# Autodesk Inventor assembly: szafa xD
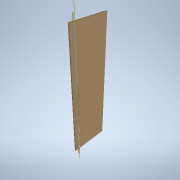
[picture p0: Inventor's stored thumbnail of the model, 180x180]
Saved by Autodesk Inventor 2021 (Build 250183000, 183)
## iProperties
Created: 2021-04-01
Part Number: szafa xD
Document SubType Name: Assembly
Designer: Wojciech Wołczek
Author: Wojciech Wołczek
## Documents named in this file (22)
- D:\OneDrive\Documents\inventor\szafa xD.iam
- D:\OneDrive\Documents\inventor\ISO 10799-2 - 25x25x2.5 - 2000.ipt
- D:\OneDrive\Documents\inventor\sciana.ipt
- D:\Documents\Inventor\Content Center Files\R2021\pl-PL\ANSI_ASME B18.6.5M(7)\ANSI_ASME B18.6.5M - M2,5x0,45 x 4(2) F.ipt
- D:\OneDrive\Documents\inventor\szafa xD\AIP\FEA\dka5v7oqo.fins
- D:\OneDrive\Documents\inventor\szafa xD\AIP\FEA\dka5v7oqo.fsat
- D:\OneDrive\Documents\inventor\szafa xD\AIP\FEA\dka5v7oqo.ftes
- D:\OneDrive\Documents\inventor\szafa xD\AIP\FEA\dka5v7oqo.fwiz
- D:\OneDrive\Documents\inventor\szafa xD\AIP\FEA\dka5v7oqp.fins
- D:\OneDrive\Documents\inventor\szafa xD\AIP\FEA\dka5v7oqp.fsat
- D:\OneDrive\Documents\inventor\szafa xD\AIP\FEA\dka5v7oqp.ftes
- D:\OneDrive\Documents\inventor\szafa xD\AIP\FEA\dka5v7oqp.fwiz
- D:\OneDrive\Documents\inventor\szafa xD\AIP\FEA\dka5v7oqq.fins
- D:\OneDrive\Documents\inventor\szafa xD\AIP\FEA\dka5v7oqq.fsat
- D:\OneDrive\Documents\inventor\szafa xD\AIP\FEA\dka5v7oqq.ftes
- D:\OneDrive\Documents\inventor\szafa xD\AIP\FEA\dka5v7ork.fwiz
- D:\OneDrive\Documents\inventor\szafa xD\AIP\FEA\dka5v7osg.fmsh
- D:\OneDrive\Documents\inventor\szafa xD\AIP\FEA\dka5v7osh.fres
- D:\OneDrive\Documents\inventor\szafa xD\AIP\FEA\dka5v7otc.fmsh
- D:\OneDrive\Documents\inventor\szafa xD\AIP\FEA\dka5v7otd.fres
- D:\OneDrive\Documents\inventor\szafa xD\AIP\FEA\dka5v7ou8.fmsh
- D:\OneDrive\Documents\inventor\szafa xD\AIP\FEA\dka5v7ou9.fres
## Components (78 placed, 3 different names)
1. ISO 10799-2 - 25x25x2.5 - 2000:1 — Równoległe:1, Równoległe:2, Wstawiające:1, Wstawiające:2, Wstawiające:3, Wstawiające:4, Wstawiające:5, Wstawiające:6, Wstawiające:7, Wstawiające:8, Wstawiające:9, Wstawiające:10, Wstawiające:11, Wstawiające:12, Wstawiające:13, Wstawiające:14, Wstawiające:15, Wstawiające:16, Wstawiające:17, Wstawiające:18, Wstawiające:19, Wstawiające:20, Wstawiające:21, Wstawiające:22, Wstawiające:23, Wstawiające:24, Wstawiające:25, Wstawiające:26, Wstawiające:27, Wstawiające:28, Wstawiające:29, Wstawiające:30, Wstawiające:31, Wstawiające:32, Wstawiające:33, Wstawiające:34, Wstawiające:35, Wstawiające:36, Wstawiające:37, Wstawiające:38, Wstawiające:39, Wstawiające:40, Wstawiające:41, Wstawiające:42, Wstawiające:43, Wstawiające:44, Wstawiające:45, Wstawiające:46, Wstawiające:47, Wstawiające:48, Wstawiające:49, Wstawiające:50, Wstawiające:51, Wstawiające:52, Wstawiające:53, Wstawiające:54, Wstawiające:55, Wstawiające:56, Wstawiające:57, Wstawiające:58, Wstawiające:59, Wstawiające:60, Wstawiające:61, Wstawiające:62, Wstawiające:63, Wstawiające:64, Wstawiające:65, Wstawiające:66, Wstawiające:67, Wstawiające:68, Wstawiające:69, Wstawiające:70, Wstawiające:71, Wstawiające:72, Wstawiające:73, Wstawiające:74, Wstawiające:75, Wstawiające:76
2. sciana:1 — Równoległe:1, Równoległe:2
3. Wkręt samogwintujący z łbem walcowym wypukłym z rowkiem prostym - Typ F - Metryczny M2,5x0,45 x 4:1 — Wstawiające:1
4. Wkręt samogwintujący z łbem walcowym wypukłym z rowkiem prostym - Typ F - Metryczny M2,5x0,45 x 4:2 — Wstawiające:2
5. Wkręt samogwintujący z łbem walcowym wypukłym z rowkiem prostym - Typ F - Metryczny M2,5x0,45 x 4:3 — Wstawiające:3
6. Wkręt samogwintujący z łbem walcowym wypukłym z rowkiem prostym - Typ F - Metryczny M2,5x0,45 x 4:4 — Wstawiające:4
7. Wkręt samogwintujący z łbem walcowym wypukłym z rowkiem prostym - Typ F - Metryczny M2,5x0,45 x 4:5 — Wstawiające:5
8. Wkręt samogwintujący z łbem walcowym wypukłym z rowkiem prostym - Typ F - Metryczny M2,5x0,45 x 4:6 — Wstawiające:6
9. Wkręt samogwintujący z łbem walcowym wypukłym z rowkiem prostym - Typ F - Metryczny M2,5x0,45 x 4:7 — Wstawiające:7
10. Wkręt samogwintujący z łbem walcowym wypukłym z rowkiem prostym - Typ F - Metryczny M2,5x0,45 x 4:8 — Wstawiające:8
11. Wkręt samogwintujący z łbem walcowym wypukłym z rowkiem prostym - Typ F - Metryczny M2,5x0,45 x 4:9 — Wstawiające:9
12. Wkręt samogwintujący z łbem walcowym wypukłym z rowkiem prostym - Typ F - Metryczny M2,5x0,45 x 4:10 — Wstawiające:10
13. Wkręt samogwintujący z łbem walcowym wypukłym z rowkiem prostym - Typ F - Metryczny M2,5x0,45 x 4:11 — Wstawiające:11
14. Wkręt samogwintujący z łbem walcowym wypukłym z rowkiem prostym - Typ F - Metryczny M2,5x0,45 x 4:12 — Wstawiające:12
15. Wkręt samogwintujący z łbem walcowym wypukłym z rowkiem prostym - Typ F - Metryczny M2,5x0,45 x 4:13 — Wstawiające:13
16. Wkręt samogwintujący z łbem walcowym wypukłym z rowkiem prostym - Typ F - Metryczny M2,5x0,45 x 4:14 — Wstawiające:14
17. Wkręt samogwintujący z łbem walcowym wypukłym z rowkiem prostym - Typ F - Metryczny M2,5x0,45 x 4:15 — Wstawiające:15
18. Wkręt samogwintujący z łbem walcowym wypukłym z rowkiem prostym - Typ F - Metryczny M2,5x0,45 x 4:16 — Wstawiające:16
19. Wkręt samogwintujący z łbem walcowym wypukłym z rowkiem prostym - Typ F - Metryczny M2,5x0,45 x 4:17 — Wstawiające:17
20. Wkręt samogwintujący z łbem walcowym wypukłym z rowkiem prostym - Typ F - Metryczny M2,5x0,45 x 4:18 — Wstawiające:18
21. Wkręt samogwintujący z łbem walcowym wypukłym z rowkiem prostym - Typ F - Metryczny M2,5x0,45 x 4:19 — Wstawiające:19
22. Wkręt samogwintujący z łbem walcowym wypukłym z rowkiem prostym - Typ F - Metryczny M2,5x0,45 x 4:20 — Wstawiające:20
23. Wkręt samogwintujący z łbem walcowym wypukłym z rowkiem prostym - Typ F - Metryczny M2,5x0,45 x 4:21 — Wstawiające:21
24. Wkręt samogwintujący z łbem walcowym wypukłym z rowkiem prostym - Typ F - Metryczny M2,5x0,45 x 4:22 — Wstawiające:22
25. Wkręt samogwintujący z łbem walcowym wypukłym z rowkiem prostym - Typ F - Metryczny M2,5x0,45 x 4:23 — Wstawiające:23
26. Wkręt samogwintujący z łbem walcowym wypukłym z rowkiem prostym - Typ F - Metryczny M2,5x0,45 x 4:24 — Wstawiające:24
27. Wkręt samogwintujący z łbem walcowym wypukłym z rowkiem prostym - Typ F - Metryczny M2,5x0,45 x 4:25 — Wstawiające:25
28. Wkręt samogwintujący z łbem walcowym wypukłym z rowkiem prostym - Typ F - Metryczny M2,5x0,45 x 4:26 — Wstawiające:26
29. Wkręt samogwintujący z łbem walcowym wypukłym z rowkiem prostym - Typ F - Metryczny M2,5x0,45 x 4:27 — Wstawiające:27
30. Wkręt samogwintujący z łbem walcowym wypukłym z rowkiem prostym - Typ F - Metryczny M2,5x0,45 x 4:28 — Wstawiające:28
31. Wkręt samogwintujący z łbem walcowym wypukłym z rowkiem prostym - Typ F - Metryczny M2,5x0,45 x 4:29 — Wstawiające:29
32. Wkręt samogwintujący z łbem walcowym wypukłym z rowkiem prostym - Typ F - Metryczny M2,5x0,45 x 4:30 — Wstawiające:30
33. Wkręt samogwintujący z łbem walcowym wypukłym z rowkiem prostym - Typ F - Metryczny M2,5x0,45 x 4:31 — Wstawiające:31
34. Wkręt samogwintujący z łbem walcowym wypukłym z rowkiem prostym - Typ F - Metryczny M2,5x0,45 x 4:32 — Wstawiające:32
35. Wkręt samogwintujący z łbem walcowym wypukłym z rowkiem prostym - Typ F - Metryczny M2,5x0,45 x 4:33 — Wstawiające:33
36. Wkręt samogwintujący z łbem walcowym wypukłym z rowkiem prostym - Typ F - Metryczny M2,5x0,45 x 4:34 — Wstawiające:34
37. Wkręt samogwintujący z łbem walcowym wypukłym z rowkiem prostym - Typ F - Metryczny M2,5x0,45 x 4:35 — Wstawiające:35
38. Wkręt samogwintujący z łbem walcowym wypukłym z rowkiem prostym - Typ F - Metryczny M2,5x0,45 x 4:36 — Wstawiające:36
39. Wkręt samogwintujący z łbem walcowym wypukłym z rowkiem prostym - Typ F - Metryczny M2,5x0,45 x 4:37 — Wstawiające:37
40. Wkręt samogwintujący z łbem walcowym wypukłym z rowkiem prostym - Typ F - Metryczny M2,5x0,45 x 4:38 — Wstawiające:38
41. Wkręt samogwintujący z łbem walcowym wypukłym z rowkiem prostym - Typ F - Metryczny M2,5x0,45 x 4:39 — Wstawiające:39
42. Wkręt samogwintujący z łbem walcowym wypukłym z rowkiem prostym - Typ F - Metryczny M2,5x0,45 x 4:40 — Wstawiające:40
43. Wkręt samogwintujący z łbem walcowym wypukłym z rowkiem prostym - Typ F - Metryczny M2,5x0,45 x 4:41 — Wstawiające:41
44. Wkręt samogwintujący z łbem walcowym wypukłym z rowkiem prostym - Typ F - Metryczny M2,5x0,45 x 4:42 — Wstawiające:42
45. Wkręt samogwintujący z łbem walcowym wypukłym z rowkiem prostym - Typ F - Metryczny M2,5x0,45 x 4:43 — Wstawiające:43
46. Wkręt samogwintujący z łbem walcowym wypukłym z rowkiem prostym - Typ F - Metryczny M2,5x0,45 x 4:44 — Wstawiające:44
47. Wkręt samogwintujący z łbem walcowym wypukłym z rowkiem prostym - Typ F - Metryczny M2,5x0,45 x 4:45 — Wstawiające:45
48. Wkręt samogwintujący z łbem walcowym wypukłym z rowkiem prostym - Typ F - Metryczny M2,5x0,45 x 4:46 — Wstawiające:46
49. Wkręt samogwintujący z łbem walcowym wypukłym z rowkiem prostym - Typ F - Metryczny M2,5x0,45 x 4:47 — Wstawiające:47
50. Wkręt samogwintujący z łbem walcowym wypukłym z rowkiem prostym - Typ F - Metryczny M2,5x0,45 x 4:48 — Wstawiające:48
51. Wkręt samogwintujący z łbem walcowym wypukłym z rowkiem prostym - Typ F - Metryczny M2,5x0,45 x 4:49 — Wstawiające:49
52. Wkręt samogwintujący z łbem walcowym wypukłym z rowkiem prostym - Typ F - Metryczny M2,5x0,45 x 4:50 — Wstawiające:50
53. Wkręt samogwintujący z łbem walcowym wypukłym z rowkiem prostym - Typ F - Metryczny M2,5x0,45 x 4:51 — Wstawiające:51
54. Wkręt samogwintujący z łbem walcowym wypukłym z rowkiem prostym - Typ F - Metryczny M2,5x0,45 x 4:52 — Wstawiające:52
55. Wkręt samogwintujący z łbem walcowym wypukłym z rowkiem prostym - Typ F - Metryczny M2,5x0,45 x 4:53 — Wstawiające:53
56. Wkręt samogwintujący z łbem walcowym wypukłym z rowkiem prostym - Typ F - Metryczny M2,5x0,45 x 4:54 — Wstawiające:54
57. Wkręt samogwintujący z łbem walcowym wypukłym z rowkiem prostym - Typ F - Metryczny M2,5x0,45 x 4:55 — Wstawiające:55
58. Wkręt samogwintujący z łbem walcowym wypukłym z rowkiem prostym - Typ F - Metryczny M2,5x0,45 x 4:56 — Wstawiające:56
59. Wkręt samogwintujący z łbem walcowym wypukłym z rowkiem prostym - Typ F - Metryczny M2,5x0,45 x 4:57 — Wstawiające:57
60. Wkręt samogwintujący z łbem walcowym wypukłym z rowkiem prostym - Typ F - Metryczny M2,5x0,45 x 4:58 — Wstawiające:58
61. Wkręt samogwintujący z łbem walcowym wypukłym z rowkiem prostym - Typ F - Metryczny M2,5x0,45 x 4:59 — Wstawiające:59
62. Wkręt samogwintujący z łbem walcowym wypukłym z rowkiem prostym - Typ F - Metryczny M2,5x0,45 x 4:60 — Wstawiające:60
63. Wkręt samogwintujący z łbem walcowym wypukłym z rowkiem prostym - Typ F - Metryczny M2,5x0,45 x 4:61 — Wstawiające:61
64. Wkręt samogwintujący z łbem walcowym wypukłym z rowkiem prostym - Typ F - Metryczny M2,5x0,45 x 4:62 — Wstawiające:62
65. Wkręt samogwintujący z łbem walcowym wypukłym z rowkiem prostym - Typ F - Metryczny M2,5x0,45 x 4:63 — Wstawiające:63
66. Wkręt samogwintujący z łbem walcowym wypukłym z rowkiem prostym - Typ F - Metryczny M2,5x0,45 x 4:64 — Wstawiające:64
67. Wkręt samogwintujący z łbem walcowym wypukłym z rowkiem prostym - Typ F - Metryczny M2,5x0,45 x 4:65 — Wstawiające:65
68. Wkręt samogwintujący z łbem walcowym wypukłym z rowkiem prostym - Typ F - Metryczny M2,5x0,45 x 4:66 — Wstawiające:66
69. Wkręt samogwintujący z łbem walcowym wypukłym z rowkiem prostym - Typ F - Metryczny M2,5x0,45 x 4:67 — Wstawiające:67
70. Wkręt samogwintujący z łbem walcowym wypukłym z rowkiem prostym - Typ F - Metryczny M2,5x0,45 x 4:68 — Wstawiające:68
71. Wkręt samogwintujący z łbem walcowym wypukłym z rowkiem prostym - Typ F - Metryczny M2,5x0,45 x 4:69 — Wstawiające:69
72. Wkręt samogwintujący z łbem walcowym wypukłym z rowkiem prostym - Typ F - Metryczny M2,5x0,45 x 4:70 — Wstawiające:70
73. Wkręt samogwintujący z łbem walcowym wypukłym z rowkiem prostym - Typ F - Metryczny M2,5x0,45 x 4:71 — Wstawiające:71
74. Wkręt samogwintujący z łbem walcowym wypukłym z rowkiem prostym - Typ F - Metryczny M2,5x0,45 x 4:72 — Wstawiające:72
75. Wkręt samogwintujący z łbem walcowym wypukłym z rowkiem prostym - Typ F - Metryczny M2,5x0,45 x 4:73 — Wstawiające:73
76. Wkręt samogwintujący z łbem walcowym wypukłym z rowkiem prostym - Typ F - Metryczny M2,5x0,45 x 4:74 — Wstawiające:74
77. Wkręt samogwintujący z łbem walcowym wypukłym z rowkiem prostym - Typ F - Metryczny M2,5x0,45 x 4:75 — Wstawiające:75
78. Wkręt samogwintujący z łbem walcowym wypukłym z rowkiem prostym - Typ F - Metryczny M2,5x0,45 x 4:76 — Wstawiające:76
## Relationships (78: Insert 76, Flush 2)
- Równoległe:1 [Flush]: ISO 10799-2 - 25x25x2.5 - 2000:1 ↔ sciana:1
- Równoległe:2 [Flush]: ISO 10799-2 - 25x25x2.5 - 2000:1 ↔ sciana:1
- Wstawiające:1 [Insert]: ISO 10799-2 - 25x25x2.5 - 2000:1 ↔ Wkręt samogwintujący z łbem walcowym wypukłym z rowkiem prostym - Typ F - Metryczny M2,5x0,45 x 4:1
- Wstawiające:2 [Insert]: ISO 10799-2 - 25x25x2.5 - 2000:1 ↔ Wkręt samogwintujący z łbem walcowym wypukłym z rowkiem prostym - Typ F - Metryczny M2,5x0,45 x 4:2
- Wstawiające:3 [Insert]: ISO 10799-2 - 25x25x2.5 - 2000:1 ↔ Wkręt samogwintujący z łbem walcowym wypukłym z rowkiem prostym - Typ F - Metryczny M2,5x0,45 x 4:3
- Wstawiające:4 [Insert]: ISO 10799-2 - 25x25x2.5 - 2000:1 ↔ Wkręt samogwintujący z łbem walcowym wypukłym z rowkiem prostym - Typ F - Metryczny M2,5x0,45 x 4:4
- Wstawiające:5 [Insert]: ISO 10799-2 - 25x25x2.5 - 2000:1 ↔ Wkręt samogwintujący z łbem walcowym wypukłym z rowkiem prostym - Typ F - Metryczny M2,5x0,45 x 4:5
- Wstawiające:6 [Insert]: ISO 10799-2 - 25x25x2.5 - 2000:1 ↔ Wkręt samogwintujący z łbem walcowym wypukłym z rowkiem prostym - Typ F - Metryczny M2,5x0,45 x 4:6
- Wstawiające:7 [Insert]: ISO 10799-2 - 25x25x2.5 - 2000:1 ↔ Wkręt samogwintujący z łbem walcowym wypukłym z rowkiem prostym - Typ F - Metryczny M2,5x0,45 x 4:7
- Wstawiające:8 [Insert]: ISO 10799-2 - 25x25x2.5 - 2000:1 ↔ Wkręt samogwintujący z łbem walcowym wypukłym z rowkiem prostym - Typ F - Metryczny M2,5x0,45 x 4:8
- Wstawiające:9 [Insert]: ISO 10799-2 - 25x25x2.5 - 2000:1 ↔ Wkręt samogwintujący z łbem walcowym wypukłym z rowkiem prostym - Typ F - Metryczny M2,5x0,45 x 4:9
- Wstawiające:10 [Insert]: ISO 10799-2 - 25x25x2.5 - 2000:1 ↔ Wkręt samogwintujący z łbem walcowym wypukłym z rowkiem prostym - Typ F - Metryczny M2,5x0,45 x 4:10
- Wstawiające:11 [Insert]: ISO 10799-2 - 25x25x2.5 - 2000:1 ↔ Wkręt samogwintujący z łbem walcowym wypukłym z rowkiem prostym - Typ F - Metryczny M2,5x0,45 x 4:11
- Wstawiające:12 [Insert]: ISO 10799-2 - 25x25x2.5 - 2000:1 ↔ Wkręt samogwintujący z łbem walcowym wypukłym z rowkiem prostym - Typ F - Metryczny M2,5x0,45 x 4:12
- Wstawiające:13 [Insert]: ISO 10799-2 - 25x25x2.5 - 2000:1 ↔ Wkręt samogwintujący z łbem walcowym wypukłym z rowkiem prostym - Typ F - Metryczny M2,5x0,45 x 4:13
- Wstawiające:14 [Insert]: ISO 10799-2 - 25x25x2.5 - 2000:1 ↔ Wkręt samogwintujący z łbem walcowym wypukłym z rowkiem prostym - Typ F - Metryczny M2,5x0,45 x 4:14
- Wstawiające:15 [Insert]: ISO 10799-2 - 25x25x2.5 - 2000:1 ↔ Wkręt samogwintujący z łbem walcowym wypukłym z rowkiem prostym - Typ F - Metryczny M2,5x0,45 x 4:15
- Wstawiające:16 [Insert]: ISO 10799-2 - 25x25x2.5 - 2000:1 ↔ Wkręt samogwintujący z łbem walcowym wypukłym z rowkiem prostym - Typ F - Metryczny M2,5x0,45 x 4:16
- Wstawiające:17 [Insert]: ISO 10799-2 - 25x25x2.5 - 2000:1 ↔ Wkręt samogwintujący z łbem walcowym wypukłym z rowkiem prostym - Typ F - Metryczny M2,5x0,45 x 4:17
- Wstawiające:18 [Insert]: ISO 10799-2 - 25x25x2.5 - 2000:1 ↔ Wkręt samogwintujący z łbem walcowym wypukłym z rowkiem prostym - Typ F - Metryczny M2,5x0,45 x 4:18
- Wstawiające:19 [Insert]: ISO 10799-2 - 25x25x2.5 - 2000:1 ↔ Wkręt samogwintujący z łbem walcowym wypukłym z rowkiem prostym - Typ F - Metryczny M2,5x0,45 x 4:19
- Wstawiające:20 [Insert]: ISO 10799-2 - 25x25x2.5 - 2000:1 ↔ Wkręt samogwintujący z łbem walcowym wypukłym z rowkiem prostym - Typ F - Metryczny M2,5x0,45 x 4:20
- Wstawiające:21 [Insert]: ISO 10799-2 - 25x25x2.5 - 2000:1 ↔ Wkręt samogwintujący z łbem walcowym wypukłym z rowkiem prostym - Typ F - Metryczny M2,5x0,45 x 4:21
- Wstawiające:22 [Insert]: ISO 10799-2 - 25x25x2.5 - 2000:1 ↔ Wkręt samogwintujący z łbem walcowym wypukłym z rowkiem prostym - Typ F - Metryczny M2,5x0,45 x 4:22
- Wstawiające:23 [Insert]: ISO 10799-2 - 25x25x2.5 - 2000:1 ↔ Wkręt samogwintujący z łbem walcowym wypukłym z rowkiem prostym - Typ F - Metryczny M2,5x0,45 x 4:23
- Wstawiające:24 [Insert]: ISO 10799-2 - 25x25x2.5 - 2000:1 ↔ Wkręt samogwintujący z łbem walcowym wypukłym z rowkiem prostym - Typ F - Metryczny M2,5x0,45 x 4:24
- Wstawiające:25 [Insert]: ISO 10799-2 - 25x25x2.5 - 2000:1 ↔ Wkręt samogwintujący z łbem walcowym wypukłym z rowkiem prostym - Typ F - Metryczny M2,5x0,45 x 4:25
- Wstawiające:26 [Insert]: ISO 10799-2 - 25x25x2.5 - 2000:1 ↔ Wkręt samogwintujący z łbem walcowym wypukłym z rowkiem prostym - Typ F - Metryczny M2,5x0,45 x 4:26
- Wstawiające:27 [Insert]: ISO 10799-2 - 25x25x2.5 - 2000:1 ↔ Wkręt samogwintujący z łbem walcowym wypukłym z rowkiem prostym - Typ F - Metryczny M2,5x0,45 x 4:27
- Wstawiające:28 [Insert]: ISO 10799-2 - 25x25x2.5 - 2000:1 ↔ Wkręt samogwintujący z łbem walcowym wypukłym z rowkiem prostym - Typ F - Metryczny M2,5x0,45 x 4:28
- Wstawiające:29 [Insert]: ISO 10799-2 - 25x25x2.5 - 2000:1 ↔ Wkręt samogwintujący z łbem walcowym wypukłym z rowkiem prostym - Typ F - Metryczny M2,5x0,45 x 4:29
- Wstawiające:30 [Insert]: ISO 10799-2 - 25x25x2.5 - 2000:1 ↔ Wkręt samogwintujący z łbem walcowym wypukłym z rowkiem prostym - Typ F - Metryczny M2,5x0,45 x 4:30
- Wstawiające:31 [Insert]: ISO 10799-2 - 25x25x2.5 - 2000:1 ↔ Wkręt samogwintujący z łbem walcowym wypukłym z rowkiem prostym - Typ F - Metryczny M2,5x0,45 x 4:31
- Wstawiające:32 [Insert]: ISO 10799-2 - 25x25x2.5 - 2000:1 ↔ Wkręt samogwintujący z łbem walcowym wypukłym z rowkiem prostym - Typ F - Metryczny M2,5x0,45 x 4:32
- Wstawiające:33 [Insert]: ISO 10799-2 - 25x25x2.5 - 2000:1 ↔ Wkręt samogwintujący z łbem walcowym wypukłym z rowkiem prostym - Typ F - Metryczny M2,5x0,45 x 4:33
- Wstawiające:34 [Insert]: ISO 10799-2 - 25x25x2.5 - 2000:1 ↔ Wkręt samogwintujący z łbem walcowym wypukłym z rowkiem prostym - Typ F - Metryczny M2,5x0,45 x 4:34
- Wstawiające:35 [Insert]: ISO 10799-2 - 25x25x2.5 - 2000:1 ↔ Wkręt samogwintujący z łbem walcowym wypukłym z rowkiem prostym - Typ F - Metryczny M2,5x0,45 x 4:35
- Wstawiające:36 [Insert]: ISO 10799-2 - 25x25x2.5 - 2000:1 ↔ Wkręt samogwintujący z łbem walcowym wypukłym z rowkiem prostym - Typ F - Metryczny M2,5x0,45 x 4:36
- Wstawiające:37 [Insert]: ISO 10799-2 - 25x25x2.5 - 2000:1 ↔ Wkręt samogwintujący z łbem walcowym wypukłym z rowkiem prostym - Typ F - Metryczny M2,5x0,45 x 4:37
- Wstawiające:38 [Insert]: ISO 10799-2 - 25x25x2.5 - 2000:1 ↔ Wkręt samogwintujący z łbem walcowym wypukłym z rowkiem prostym - Typ F - Metryczny M2,5x0,45 x 4:38
- Wstawiające:39 [Insert]: ISO 10799-2 - 25x25x2.5 - 2000:1 ↔ Wkręt samogwintujący z łbem walcowym wypukłym z rowkiem prostym - Typ F - Metryczny M2,5x0,45 x 4:39
- Wstawiające:40 [Insert]: ISO 10799-2 - 25x25x2.5 - 2000:1 ↔ Wkręt samogwintujący z łbem walcowym wypukłym z rowkiem prostym - Typ F - Metryczny M2,5x0,45 x 4:40
- Wstawiające:41 [Insert]: ISO 10799-2 - 25x25x2.5 - 2000:1 ↔ Wkręt samogwintujący z łbem walcowym wypukłym z rowkiem prostym - Typ F - Metryczny M2,5x0,45 x 4:41
- Wstawiające:42 [Insert]: ISO 10799-2 - 25x25x2.5 - 2000:1 ↔ Wkręt samogwintujący z łbem walcowym wypukłym z rowkiem prostym - Typ F - Metryczny M2,5x0,45 x 4:42
- Wstawiające:43 [Insert]: ISO 10799-2 - 25x25x2.5 - 2000:1 ↔ Wkręt samogwintujący z łbem walcowym wypukłym z rowkiem prostym - Typ F - Metryczny M2,5x0,45 x 4:43
- Wstawiające:44 [Insert]: ISO 10799-2 - 25x25x2.5 - 2000:1 ↔ Wkręt samogwintujący z łbem walcowym wypukłym z rowkiem prostym - Typ F - Metryczny M2,5x0,45 x 4:44
- Wstawiające:45 [Insert]: ISO 10799-2 - 25x25x2.5 - 2000:1 ↔ Wkręt samogwintujący z łbem walcowym wypukłym z rowkiem prostym - Typ F - Metryczny M2,5x0,45 x 4:45
- Wstawiające:46 [Insert]: ISO 10799-2 - 25x25x2.5 - 2000:1 ↔ Wkręt samogwintujący z łbem walcowym wypukłym z rowkiem prostym - Typ F - Metryczny M2,5x0,45 x 4:46
- Wstawiające:47 [Insert]: ISO 10799-2 - 25x25x2.5 - 2000:1 ↔ Wkręt samogwintujący z łbem walcowym wypukłym z rowkiem prostym - Typ F - Metryczny M2,5x0,45 x 4:47
- Wstawiające:48 [Insert]: ISO 10799-2 - 25x25x2.5 - 2000:1 ↔ Wkręt samogwintujący z łbem walcowym wypukłym z rowkiem prostym - Typ F - Metryczny M2,5x0,45 x 4:48
- Wstawiające:49 [Insert]: ISO 10799-2 - 25x25x2.5 - 2000:1 ↔ Wkręt samogwintujący z łbem walcowym wypukłym z rowkiem prostym - Typ F - Metryczny M2,5x0,45 x 4:49
- Wstawiające:50 [Insert]: ISO 10799-2 - 25x25x2.5 - 2000:1 ↔ Wkręt samogwintujący z łbem walcowym wypukłym z rowkiem prostym - Typ F - Metryczny M2,5x0,45 x 4:50
- Wstawiające:51 [Insert]: ISO 10799-2 - 25x25x2.5 - 2000:1 ↔ Wkręt samogwintujący z łbem walcowym wypukłym z rowkiem prostym - Typ F - Metryczny M2,5x0,45 x 4:51
- Wstawiające:52 [Insert]: ISO 10799-2 - 25x25x2.5 - 2000:1 ↔ Wkręt samogwintujący z łbem walcowym wypukłym z rowkiem prostym - Typ F - Metryczny M2,5x0,45 x 4:52
- Wstawiające:53 [Insert]: ISO 10799-2 - 25x25x2.5 - 2000:1 ↔ Wkręt samogwintujący z łbem walcowym wypukłym z rowkiem prostym - Typ F - Metryczny M2,5x0,45 x 4:53
- Wstawiające:54 [Insert]: ISO 10799-2 - 25x25x2.5 - 2000:1 ↔ Wkręt samogwintujący z łbem walcowym wypukłym z rowkiem prostym - Typ F - Metryczny M2,5x0,45 x 4:54
- Wstawiające:55 [Insert]: ISO 10799-2 - 25x25x2.5 - 2000:1 ↔ Wkręt samogwintujący z łbem walcowym wypukłym z rowkiem prostym - Typ F - Metryczny M2,5x0,45 x 4:55
- Wstawiające:56 [Insert]: ISO 10799-2 - 25x25x2.5 - 2000:1 ↔ Wkręt samogwintujący z łbem walcowym wypukłym z rowkiem prostym - Typ F - Metryczny M2,5x0,45 x 4:56
- Wstawiające:57 [Insert]: ISO 10799-2 - 25x25x2.5 - 2000:1 ↔ Wkręt samogwintujący z łbem walcowym wypukłym z rowkiem prostym - Typ F - Metryczny M2,5x0,45 x 4:57
- Wstawiające:58 [Insert]: ISO 10799-2 - 25x25x2.5 - 2000:1 ↔ Wkręt samogwintujący z łbem walcowym wypukłym z rowkiem prostym - Typ F - Metryczny M2,5x0,45 x 4:58
- Wstawiające:59 [Insert]: ISO 10799-2 - 25x25x2.5 - 2000:1 ↔ Wkręt samogwintujący z łbem walcowym wypukłym z rowkiem prostym - Typ F - Metryczny M2,5x0,45 x 4:59
- Wstawiające:60 [Insert]: ISO 10799-2 - 25x25x2.5 - 2000:1 ↔ Wkręt samogwintujący z łbem walcowym wypukłym z rowkiem prostym - Typ F - Metryczny M2,5x0,45 x 4:60
- Wstawiające:61 [Insert]: ISO 10799-2 - 25x25x2.5 - 2000:1 ↔ Wkręt samogwintujący z łbem walcowym wypukłym z rowkiem prostym - Typ F - Metryczny M2,5x0,45 x 4:61
- Wstawiające:62 [Insert]: ISO 10799-2 - 25x25x2.5 - 2000:1 ↔ Wkręt samogwintujący z łbem walcowym wypukłym z rowkiem prostym - Typ F - Metryczny M2,5x0,45 x 4:62
- Wstawiające:63 [Insert]: ISO 10799-2 - 25x25x2.5 - 2000:1 ↔ Wkręt samogwintujący z łbem walcowym wypukłym z rowkiem prostym - Typ F - Metryczny M2,5x0,45 x 4:63
- Wstawiające:64 [Insert]: ISO 10799-2 - 25x25x2.5 - 2000:1 ↔ Wkręt samogwintujący z łbem walcowym wypukłym z rowkiem prostym - Typ F - Metryczny M2,5x0,45 x 4:64
- Wstawiające:65 [Insert]: ISO 10799-2 - 25x25x2.5 - 2000:1 ↔ Wkręt samogwintujący z łbem walcowym wypukłym z rowkiem prostym - Typ F - Metryczny M2,5x0,45 x 4:65
- Wstawiające:66 [Insert]: ISO 10799-2 - 25x25x2.5 - 2000:1 ↔ Wkręt samogwintujący z łbem walcowym wypukłym z rowkiem prostym - Typ F - Metryczny M2,5x0,45 x 4:66
- Wstawiające:67 [Insert]: ISO 10799-2 - 25x25x2.5 - 2000:1 ↔ Wkręt samogwintujący z łbem walcowym wypukłym z rowkiem prostym - Typ F - Metryczny M2,5x0,45 x 4:67
- Wstawiające:68 [Insert]: ISO 10799-2 - 25x25x2.5 - 2000:1 ↔ Wkręt samogwintujący z łbem walcowym wypukłym z rowkiem prostym - Typ F - Metryczny M2,5x0,45 x 4:68
- Wstawiające:69 [Insert]: ISO 10799-2 - 25x25x2.5 - 2000:1 ↔ Wkręt samogwintujący z łbem walcowym wypukłym z rowkiem prostym - Typ F - Metryczny M2,5x0,45 x 4:69
- Wstawiające:70 [Insert]: ISO 10799-2 - 25x25x2.5 - 2000:1 ↔ Wkręt samogwintujący z łbem walcowym wypukłym z rowkiem prostym - Typ F - Metryczny M2,5x0,45 x 4:70
- Wstawiające:71 [Insert]: ISO 10799-2 - 25x25x2.5 - 2000:1 ↔ Wkręt samogwintujący z łbem walcowym wypukłym z rowkiem prostym - Typ F - Metryczny M2,5x0,45 x 4:71
- Wstawiające:72 [Insert]: ISO 10799-2 - 25x25x2.5 - 2000:1 ↔ Wkręt samogwintujący z łbem walcowym wypukłym z rowkiem prostym - Typ F - Metryczny M2,5x0,45 x 4:72
- Wstawiające:73 [Insert]: ISO 10799-2 - 25x25x2.5 - 2000:1 ↔ Wkręt samogwintujący z łbem walcowym wypukłym z rowkiem prostym - Typ F - Metryczny M2,5x0,45 x 4:73
- Wstawiające:74 [Insert]: ISO 10799-2 - 25x25x2.5 - 2000:1 ↔ Wkręt samogwintujący z łbem walcowym wypukłym z rowkiem prostym - Typ F - Metryczny M2,5x0,45 x 4:74
- Wstawiające:75 [Insert]: ISO 10799-2 - 25x25x2.5 - 2000:1 ↔ Wkręt samogwintujący z łbem walcowym wypukłym z rowkiem prostym - Typ F - Metryczny M2,5x0,45 x 4:75
- Wstawiające:76 [Insert]: ISO 10799-2 - 25x25x2.5 - 2000:1 ↔ Wkręt samogwintujący z łbem walcowym wypukłym z rowkiem prostym - Typ F - Metryczny M2,5x0,45 x 4:76
## Named parameters: sa_0 = 20000, sa_1 = 20000, sa_2 = 20000
note: some values were not read from the file. Shown as the stored number, unit unknown: "sa_0", "sa_1", "sa_2".
